# Autodesk Inventor assembly: Assembly2
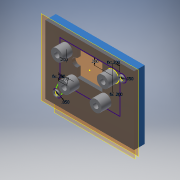
[picture p0: Inventor's stored thumbnail of the model, 180x180]
Saved by Autodesk Inventor 2017 (Build 210142000, 142)
## iProperties
Created: 2016-12-20
Part Number: Assembly2
Document SubType Name: Assembly
Designer: PLTW
Author: PLTW
## Documents named in this file (9)
- C:\Users\PLTW\Documents\Inventor\PixyCam and Gimbal\Assembly2.iam
- C:\Users\PLTW\Documents\Inventor\PixyCam and Gimbal\PixyCamKinda.ipt
- C:\Users\PLTW\Documents\Inventor\PixyCam and Gimbal\focusSpacer.ipt
- C:\Users\PLTW\Documents\Inventor\PixyCam and Gimbal\LEDRing.ipt
- C:\Users\PLTW\Documents\Inventor\PixyCam and Gimbal\backCase.ipt
- C:\Users\PLTW\Documents\Inventor\PixyCam and Gimbal\frontCase.ipt
- C:\Users\PLTW\Documents\Inventor\PixyCam and Gimbal\Ring Front.ipt
- C:\Users\PLTW\Documents\Inventor\PixyCam and Gimbal\Ring Holder.ipt
- C:\Users\PLTW\Documents\Inventor\PixyCam and Gimbal\The Holdy Thing.ipt
## Components (8 placed, 8 different names)
1. PixyCamKinda:1 — Insert:1, Insert:2, Flush:1, Flush:2, Flush:3, Flush:4
2. focusSpacer:1 — Insert:1
3. LEDRing:1 — Insert:2, Flush:6, Flush:7
4. backCase:1 — Flush:1, Flush:2, Flush:5
5. frontCase:1 — Flush:3, Flush:4, Flush:5, Flush:11, Flush:12
6. Ring Front:1 — Flush:6, Flush:7, Flush:8, Flush:9
7. Ring Holder:1 — Flush:8, Flush:9, Flush:10
8. The Holdy Thing:1 — Flush:10, Flush:11, Flush:12
## Relationships (14: Flush 12, Insert 2)
- Insert:1: PixyCamKinda:1 ↔ focusSpacer:1
- Insert:2: PixyCamKinda:1 ↔ LEDRing:1
- Flush:1: PixyCamKinda:1 ↔ backCase:1
- Flush:2: PixyCamKinda:1 ↔ backCase:1
- Flush:3: PixyCamKinda:1 ↔ frontCase:1
- Flush:4: PixyCamKinda:1 ↔ frontCase:1
- Flush:5: backCase:1 ↔ frontCase:1
- Flush:6: LEDRing:1 ↔ Ring Front:1
- Flush:7: LEDRing:1 ↔ Ring Front:1
- Flush:8: Ring Front:1 ↔ Ring Holder:1
- Flush:9: Ring Front:1 ↔ Ring Holder:1
- Flush:10: Ring Holder:1 ↔ The Holdy Thing:1
- Flush:11: frontCase:1 ↔ The Holdy Thing:1
- Flush:12: frontCase:1 ↔ The Holdy Thing:1
